# Autodesk Inventor assembly: Ensamble_Pierna
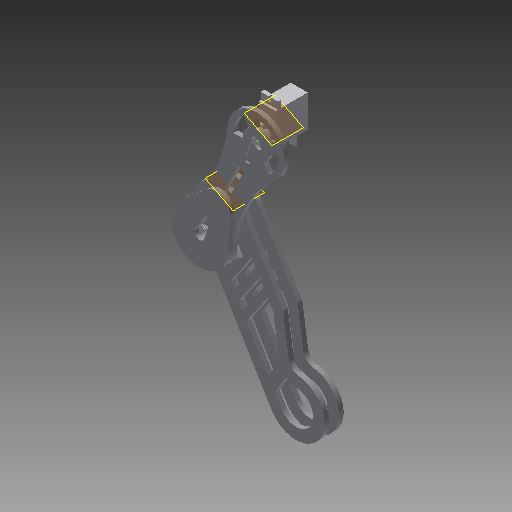
[picture p0: Inventor's stored thumbnail of the model, 512x512]
Saved by Autodesk Inventor 2019 (Build 230136000, 136)
## iProperties
Created: 2020-02-12
Part Number: Ensamble_Pierna
Document SubType Name: Assembly
Designer: jacqu
Author: jacqu
## Documents named in this file (5)
- E:\Escritorio\Temporal\Documentos\Robótica I\ProyectoCuadrupedo\Proyecto1\Proyecto1\Ensamble_Pierna.iam
- E:\Escritorio\Temporal\Documentos\Robótica I\ProyectoCuadrupedo\Proyecto1\Proyecto1\Pata - Soporte Antebrazo.ipt
- E:\Escritorio\Temporal\Documentos\Robótica I\ProyectoCuadrupedo\Proyecto1\Proyecto1\Pata - Antebrazo.ipt
- E:\Escritorio\Temporal\Documentos\Robótica I\ProyectoCuadrupedo\Proyecto1\Proyecto1\Pata - Brazo.ipt
- E:\Escritorio\Temporal\Documentos\Robótica I\ProyectoCuadrupedo\Proyecto1\Proyecto1\Servo - Componente.ipt
## Components (6 placed, 4 different names)
1. pierna1:1 — Mate:4, Mate:5, Mate:6
2. pierna1_2:1 — Mate:4, Mate:5, Mate:6, Mate:12, Mate:13, Mate:14, Mate:15
3. Pierna2:1 — Mate:1, Mate:7, Mate:8
4. servo:1 — Mate:1, Mate:7, Mate:8, Mate:9, Mate:10, Mate:11, Mate:12, Mate:13
5. servo:2 — Mate:14, Mate:15
6. Pierna2:2 — Mate:9, Mate:10, Mate:11
## Relationships (13: Mate 13)
- Mate:1: Pierna2:1 ↔ servo:1
- Mate:4: pierna1:1 ↔ pierna1_2:1
- Mate:5: pierna1:1 ↔ pierna1_2:1
- Mate:6: pierna1:1 ↔ pierna1_2:1
- Mate:7: Pierna2:1 ↔ servo:1
- Mate:8: Pierna2:1 ↔ servo:1
- Mate:9: servo:1 ↔ Pierna2:2
- Mate:10: servo:1 ↔ Pierna2:2
- Mate:11: servo:1 ↔ Pierna2:2
- Mate:12: pierna1_2:1 ↔ servo:1
- Mate:13: pierna1_2:1 ↔ servo:1
- Mate:14: pierna1_2:1 ↔ servo:2
- Mate:15: pierna1_2:1 ↔ servo:2
